# Autodesk Inventor assembly: construction
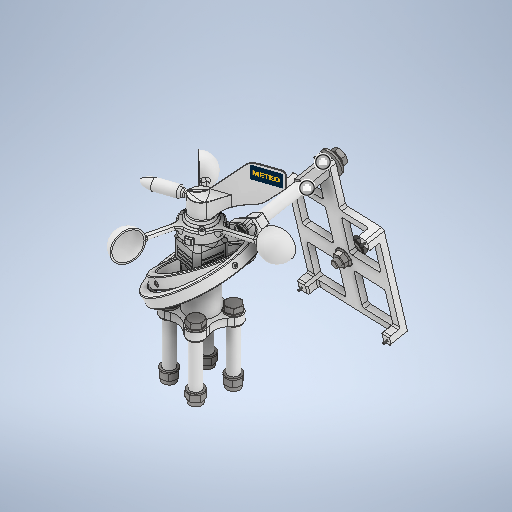
[picture p0: Inventor's stored thumbnail of the model, 512x512]
Saved by Autodesk Inventor 2025.2 (Build 292293000, 293)
## iProperties
Created: 2025-02-10
Part Number: construction
Document SubType Name: Assembly
Designer: yehorderehus
Mass: 762.848 g
Surface Area: 1512.83 cm^2
Volume: 321.338 cm^3
Density: 2.37397 g/cm^3
Author: yehorderehus
## Documents named in this file (32)
- G:\.shortcut-targets-by-id\1Afqr12NmjXaFk11r_F7oLitoDl4TiMfc\Structures\assembly\assembly.iam
- G:\.shortcut-targets-by-id\1Afqr12NmjXaFk11r_F7oLitoDl4TiMfc\Structures\assembly\base-radiator.ipt
- G:\.shortcut-targets-by-id\1Afqr12NmjXaFk11r_F7oLitoDl4TiMfc\Structures\assembly\connector-main.ipt
- G:\.shortcut-targets-by-id\1Afqr12NmjXaFk11r_F7oLitoDl4TiMfc\Structures\assembly\magnet-holder.ipt
- G:\.shortcut-targets-by-id\1Afqr12NmjXaFk11r_F7oLitoDl4TiMfc\Structures\assembly\assets\skf_bearing_623-2z_2.iam
- G:\.shortcut-targets-by-id\1Afqr12NmjXaFk11r_F7oLitoDl4TiMfc\Structures\assembly\assets\skf_bearing_608-2z_2.iam
- G:\.shortcut-targets-by-id\1Afqr12NmjXaFk11r_F7oLitoDl4TiMfc\Structures\assembly\speed-rotor.ipt
- G:\.shortcut-targets-by-id\1Afqr12NmjXaFk11r_F7oLitoDl4TiMfc\Structures\assembly\distance-ring.ipt
- G:\.shortcut-targets-by-id\1Afqr12NmjXaFk11r_F7oLitoDl4TiMfc\Structures\assembly\bearing-clamp.ipt
- G:\.shortcut-targets-by-id\1Afqr12NmjXaFk11r_F7oLitoDl4TiMfc\Structures\assembly\direction-vane.ipt
- G:\.shortcut-targets-by-id\1Afqr12NmjXaFk11r_F7oLitoDl4TiMfc\Structures\assembly\Ambient_board_Meteostanice.iam
- G:\.shortcut-targets-by-id\1Afqr12NmjXaFk11r_F7oLitoDl4TiMfc\Structures\assembly\o-ring.ipt
- G:\.shortcut-targets-by-id\1Afqr12NmjXaFk11r_F7oLitoDl4TiMfc\Structures\assembly\i-ring.ipt
- D:\Users\yehorderehus\Documents\Inventor\Content Center Files\R2025\en-US\ISO 4014(2)\ISO 4014 - M12 x 90 - ISO.ipt
- D:\Users\yehorderehus\Documents\Inventor\Content Center Files\R2025\en-US\DIN 7985 (H)\DIN 7985 (H) - M3x5-H.ipt
- D:\Users\yehorderehus\Documents\Inventor\Content Center Files\R2025\en-US\DIN 7985 (H)\DIN 7985 (H) - M3x16-H.ipt
- D:\Users\yehorderehus\Documents\Inventor\Content Center Files\R2025\en-US\SFS 2976\SFS 2976 - M3 x 40.ipt
- G:\.shortcut-targets-by-id\1Afqr12NmjXaFk11r_F7oLitoDl4TiMfc\Structures\assembly\assets\magnet5_2.ipt
- G:\.shortcut-targets-by-id\1Afqr12NmjXaFk11r_F7oLitoDl4TiMfc\Structures\assembly\assets\magnet10_5.ipt
- G:\.shortcut-targets-by-id\1Afqr12NmjXaFk11r_F7oLitoDl4TiMfc\Structures\assembly\m12-60-ring.ipt
- G:\.shortcut-targets-by-id\1Afqr12NmjXaFk11r_F7oLitoDl4TiMfc\Structures\assembly\assets\Hexagon nut DIN 6334 M10 51103_100_040(High).ipt
- G:\.shortcut-targets-by-id\1Afqr12NmjXaFk11r_F7oLitoDl4TiMfc\Structures\assembly\box-mount.ipt
- D:\Users\yehorderehus\Documents\Inventor\Content Center Files\R2025\en-US\DIN 9021\DIN 9021 - 10,5.ipt
- D:\Users\yehorderehus\Documents\Inventor\Content Center Files\R2025\en-US\DIN 128\DIN 128 - A10.ipt
- D:\Users\yehorderehus\Documents\Inventor\Content Center Files\R2025\en-US\DIN 933\DIN 933 - M10  x 30.ipt
- D:\Users\yehorderehus\Documents\Inventor\Content Center Files\R2025\en-US\ISO 7380-1\ISO 7380-1 - M10 x 90.ipt
- D:\Users\yehorderehus\Documents\Inventor\Content Center Files\R2025\en-US\DIN 6923\DIN 6923 - M10 x 1,5.ipt
- D:\Users\yehorderehus\Documents\Inventor\Content Center Files\R2025\en-US\ISO 7045  H\ISO 7045 - M3 x 25_ - 4.8 - H - ISO.ipt
- G:\.shortcut-targets-by-id\1Afqr12NmjXaFk11r_F7oLitoDl4TiMfc\Structures\assembly\m10-52-ring.ipt
- D:\Users\yehorderehus\Documents\Inventor\Content Center Files\R2025\en-US\ISO 7092\ISO 7092 - ST 12 - 140 HV.ipt
- G:\.shortcut-targets-by-id\1Afqr12NmjXaFk11r_F7oLitoDl4TiMfc\Structures\assembly\assets\insert_m3_5-7.ipt
- D:\Users\yehorderehus\Documents\Inventor\Content Center Files\R2025\en-US\ISO 10512\ISO 10512 - M12 x 1,5.ipt
## Components (81 placed, 31 different names)
1. connector-main:1 — Mate:1, Rotational:1, Flush:1, Flush:2, Rotational:10, Flush:3, Rigid:25, Rigid:4, Rotational:50, Rotational:51, Rigid:55, Rigid:56, Rigid:57, Rigid:58, Rigid:59, Rigid:60, Rigid:61, Rigid:64
2. base-radiator:1 — Rotational:1, Flush:1, Rotational:2, Rotational:4, Rotational:8, Rigid:33, Rigid:32, Rigid:31
3. magnet-holder:1 — Rotational:3, Rotational:12, Rigid:30
4. distance-ring:1 — Rotational:6, Rotational:7
5. bearing-clamp:1 — Rotational:8
6. direction-vane:1 — Rotational:9, Rigid:37
7. speed-rotor:1 — Rigid:35, Rigid:34, Rigid:36, Rigid:29, Rotational:5
8. o-ring:1 — Rigid:26, Rigid:27, Rotational:24, Rigid:62, Rigid:63
9. i-ring:1 — Rotational:25, Rigid:50, Rigid:54
10. Ambient_board_Meteostanice:1 [sub-assembly] — Rotational:10, Flush:3, Rigid:1, Rigid:2, Rigid:3
11. skf_bearing_623-2z_2:1 [sub-assembly] — Rotational:2, Rotational:3
12. skf_bearing_608-2z_2:1 [sub-assembly] — Rotational:4, Rotational:5, Rotational:6
13. skf_bearing_608-2z_2:2 [sub-assembly] — Rotational:7, Rotational:9
14. magnet10_5:1 — Rigid:30
15. SFS 2976 M3 x 40:1 — Rotational:12
16. DIN 7985 (H) M3x16-H:1 — Rigid:27
17. DIN 7985 (H) M3x16-H:2 — Rigid:26, Rotational:25
18. SFS 2976 M3 x 40:2 — Rigid:25, Rotational:24
19. SFS 2976 M3 x 40:3 — Rigid:4
20. DIN 7985 (H) M3x5-H:1 — Rigid:33
21. DIN 7985 (H) M3x5-H:2 — Rigid:32
22. DIN 7985 (H) M3x5-H:3 — Rigid:31
23. DIN 7985 (H) M3x5-H:4 — Rigid:35
24. DIN 7985 (H) M3x5-H:5 — Rigid:34
25. DIN 7985 (H) M3x5-H:6 — Rigid:36
26. DIN 7985 (H) M3x5-H:7 — Rigid:37
27. DIN 7985 (H) M3x5-H:8 — Rigid:3
28. DIN 7985 (H) M3x5-H:9 — Rigid:1
29. DIN 7985 (H) M3x5-H:10 — Rigid:2
30. ISO 7380-1 M10 x 90:1 — Rigid:50, Rigid:52
31. m10-52-ring:1 — Rigid:54
32. Hexagon nut DIN 6334 M10 51103_100_040(High):1 — Rigid:49
33. box-mount:1 — Rigid:46, Rotational:48, Rigid:49, Mate:15, Rigid:53, Angle:1
34. DIN 933 - replaced by DIN EN 24017 M10  x 30:1 — Mate:4, Mate:5, Mate:8, Rigid:52
35. DIN 9021 10,5:1 — Mate:4, Mate:5, Mate:9
36. DIN 128 A10:1 — Mate:8, Mate:9, Rotational:48
37. DIN 933 - replaced by DIN EN 24017 M10  x 30:2 — Mate:6, Mate:7, Mate:12, Mate:14
38. DIN 9021 10,5:2 — Mate:6, Mate:7, Mate:13
39. DIN 128 A10:2 — Mate:12, Mate:13, Rigid:46
40. DIN 6923 M10:1 — Mate:14, Mate:15
41. insert_m3_5-7:1 — Rigid:55
42. insert_m3_5-7:2 — Rigid:56
43. insert_m3_5-7:3 — Rigid:57
44. insert_m3_5-7:4 — Rigid:61
45. insert_m3_5-7:5 — Rigid:58
46. insert_m3_5-7:6 — Rigid:59
47. insert_m3_5-7:7 — Rigid:60
48. insert_m3_5-7:8 — Rigid:64
49. insert_m3_5-7:9 — Rigid:62
50. insert_m3_5-7:10 — Rigid:63
51. magnet5_2:1 — Rigid:29
52. magnet5_2:2
53. magnet5_2:3
54. ISO 4014 M12 x 90:5 — Rotational:49, Rotational:54
55. ISO 7092 ST 12 - 140 HV:1 — Rotational:49, Rotational:50
56. ISO 7092 ST 12 - 140 HV:2 — Rotational:51, Rotational:52
57. m12-60-ring:1 — Rotational:52, Rotational:53
58. ISO 7092 ST 12 - 140 HV:3 — Rotational:53
59. DIN EN ISO 10512 M12 x 1,5:1 — Rotational:54
60. ISO 4014 M12 x 90:6
61. ISO 7092 ST 12 - 140 HV:4
62. ISO 7092 ST 12 - 140 HV:5
63. m12-60-ring:2
64. ISO 7092 ST 12 - 140 HV:6
65. DIN EN ISO 10512 M12 x 1,5:2
66. ISO 4014 M12 x 90:7
67. ISO 7092 ST 12 - 140 HV:7
68. ISO 7092 ST 12 - 140 HV:8
69. m12-60-ring:3
70. ISO 7092 ST 12 - 140 HV:9
71. DIN EN ISO 10512 M12 x 1,5:3
72. ISO 4014 M12 x 90:8
73. ISO 7092 ST 12 - 140 HV:10
74. ISO 7092 ST 12 - 140 HV:11
75. m12-60-ring:4
76. ISO 7092 ST 12 - 140 HV:12
77. DIN EN ISO 10512 M12 x 1,5:4
78. ISO 7045 H M3 x 25 - 4.8 - H:1 — Rigid:53
79. ISO 7045 H M3 x 25 - 4.8 - H:2
80. ISO 7045 H M3 x 25 - 4.8 - H:3
81. ISO 7045 H M3 x 25 - 4.8 - H:4
## Component patterns: (3 elements, first: magnet5_2:1), (4 elements, first: ISO 4014 M12 x 90:5 + ISO 7092 ST 12 - 140 HV:1 + ISO 7092 ST 12 - 140 HV:2 + m12-60-ring:1 + ISO 7092 ST 12 - 140 HV:3 + DIN EN ISO 10512 M12 x 1,5:1), (4 elements, first: ISO 7045 H M3 x 25 - 4.8 - H:1)
## Relationships (67: WeldJoint 32, RevoluteJoint 20, Mate 11, Flush 3, Angle 1)
- Mate:1: connector-main:1
- Rotational:1 [RevoluteJoint]: connector-main:1 ↔ base-radiator:1
- Flush:1: connector-main:1 ↔ base-radiator:1
- Rotational:2 [RevoluteJoint]: base-radiator:1 ↔ skf_bearing_623-2z_2:1
- Rotational:3 [RevoluteJoint]: magnet-holder:1 ↔ skf_bearing_623-2z_2:1
- Rotational:4 [RevoluteJoint]: base-radiator:1 ↔ skf_bearing_608-2z_2:1
- Rotational:6 [RevoluteJoint]: distance-ring:1 ↔ skf_bearing_608-2z_2:1
- Rotational:7 [RevoluteJoint]: distance-ring:1 ↔ skf_bearing_608-2z_2:2
- Flush:2 (61.038 mm): connector-main:1
- Rotational:8 [RevoluteJoint]: base-radiator:1 ↔ bearing-clamp:1
- Rotational:9 [RevoluteJoint]: direction-vane:1 ↔ skf_bearing_608-2z_2:2
- Rotational:10 [RevoluteJoint]: connector-main:1 ↔ Ambient_board_Meteostanice:1
- Flush:3 (1.8 mm): connector-main:1 ↔ Ambient_board_Meteostanice:1
- Rotational:12 [RevoluteJoint]: magnet-holder:1 ↔ SFS 2976 M3 x 40:1
- Rigid:33 [WeldJoint]: base-radiator:1 ↔ DIN 7985 (H) M3x5-H:1
- Rigid:32 [WeldJoint]: base-radiator:1 ↔ DIN 7985 (H) M3x5-H:2
- Rigid:31 [WeldJoint]: base-radiator:1 ↔ DIN 7985 (H) M3x5-H:3
- Rigid:35 [WeldJoint] (0.2 mm): speed-rotor:1 ↔ DIN 7985 (H) M3x5-H:4
- Rigid:34 [WeldJoint] (0.2 mm): speed-rotor:1 ↔ DIN 7985 (H) M3x5-H:5
- Rigid:36 [WeldJoint] (0.2 mm): speed-rotor:1 ↔ DIN 7985 (H) M3x5-H:6
- Rigid:37 [WeldJoint] (0.4 mm): direction-vane:1 ↔ DIN 7985 (H) M3x5-H:7
- Rigid:1 [WeldJoint]: Ambient_board_Meteostanice:1 ↔ DIN 7985 (H) M3x5-H:9
- Rigid:2 [WeldJoint]: Ambient_board_Meteostanice:1 ↔ DIN 7985 (H) M3x5-H:10
- Rigid:3 [WeldJoint]: Ambient_board_Meteostanice:1 ↔ DIN 7985 (H) M3x5-H:8
- Rigid:25 [WeldJoint]: connector-main:1 ↔ SFS 2976 M3 x 40:2
- Rigid:4 [WeldJoint]: connector-main:1 ↔ SFS 2976 M3 x 40:3
- Rigid:26 [WeldJoint]: o-ring:1 ↔ DIN 7985 (H) M3x16-H:2
- Rigid:27 [WeldJoint]: o-ring:1 ↔ DIN 7985 (H) M3x16-H:1
- Rotational:24 [RevoluteJoint] (-0.4 mm): o-ring:1 ↔ SFS 2976 M3 x 40:2
- Rotational:25 [RevoluteJoint] (0.4 mm): i-ring:1 ↔ DIN 7985 (H) M3x16-H:2
- Rigid:29 [WeldJoint]: speed-rotor:1 ↔ magnet5_2:1
- Rotational:5 [RevoluteJoint]: speed-rotor:1 ↔ skf_bearing_608-2z_2:1
- Rigid:30 [WeldJoint]: magnet-holder:1 ↔ magnet10_5:1
- Mate:4: DIN 933 - replaced by DIN EN 24017 M10  x 30:1 ↔ DIN 9021 10,5:1
- Mate:5 (4.2 mm): DIN 933 - replaced by DIN EN 24017 M10  x 30:1 ↔ DIN 9021 10,5:1
- Mate:6: DIN 933 - replaced by DIN EN 24017 M10  x 30:2 ↔ DIN 9021 10,5:2
- Mate:7 (4.2 mm): DIN 933 - replaced by DIN EN 24017 M10  x 30:2 ↔ DIN 9021 10,5:2
- Mate:8: DIN 933 - replaced by DIN EN 24017 M10  x 30:1 ↔ DIN 128 A10:1
- Mate:9 (0.2 mm): DIN 9021 10,5:1 ↔ DIN 128 A10:1
- Mate:12: DIN 933 - replaced by DIN EN 24017 M10  x 30:2 ↔ DIN 128 A10:2
- Mate:13 (0.2 mm): DIN 9021 10,5:2 ↔ DIN 128 A10:2
- Rigid:46 [WeldJoint] (0.2 mm): box-mount:1 ↔ DIN 128 A10:2
- Rotational:48 [RevoluteJoint] (0.2 mm): box-mount:1 ↔ DIN 128 A10:1
- Rigid:49 [WeldJoint]: Hexagon nut DIN 6334 M10 51103_100_040(High):1 ↔ box-mount:1
- Rigid:50 [WeldJoint]: i-ring:1 ↔ ISO 7380-1 M10 x 90:1
- Rigid:52 [WeldJoint]: ISO 7380-1 M10 x 90:1 ↔ DIN 933 - replaced by DIN EN 24017 M10  x 30:1
- Mate:14: DIN 933 - replaced by DIN EN 24017 M10  x 30:2 ↔ DIN 6923 M10:1
- Mate:15: box-mount:1 ↔ DIN 6923 M10:1
- Rigid:53 [WeldJoint]: box-mount:1 ↔ ISO 7045 H M3 x 25 - 4.8 - H:1
- Angle:1 (-90 deg): box-mount:1
- Rigid:54 [WeldJoint]: i-ring:1 ↔ m10-52-ring:1
- Rotational:49 [RevoluteJoint]: ISO 4014 M12 x 90:5 ↔ ISO 7092 ST 12 - 140 HV:1
- Rotational:50 [RevoluteJoint]: connector-main:1 ↔ ISO 7092 ST 12 - 140 HV:1
- Rotational:51 [RevoluteJoint]: connector-main:1 ↔ ISO 7092 ST 12 - 140 HV:2
- Rotational:52 [RevoluteJoint]: ISO 7092 ST 12 - 140 HV:2 ↔ m12-60-ring:1
- Rotational:53 [RevoluteJoint]: m12-60-ring:1 ↔ ISO 7092 ST 12 - 140 HV:3
- Rotational:54 [RevoluteJoint]: ISO 4014 M12 x 90:5 ↔ DIN EN ISO 10512 M12 x 1,5:1
- Rigid:55 [WeldJoint]: connector-main:1 ↔ insert_m3_5-7:1
- Rigid:56 [WeldJoint]: connector-main:1 ↔ insert_m3_5-7:2
- Rigid:57 [WeldJoint]: connector-main:1 ↔ insert_m3_5-7:3
- Rigid:58 [WeldJoint]: connector-main:1 ↔ insert_m3_5-7:5
- Rigid:59 [WeldJoint]: connector-main:1 ↔ insert_m3_5-7:6
- Rigid:60 [WeldJoint]: connector-main:1 ↔ insert_m3_5-7:7
- Rigid:61 [WeldJoint]: connector-main:1 ↔ insert_m3_5-7:4
- Rigid:62 [WeldJoint]: o-ring:1 ↔ insert_m3_5-7:9
- Rigid:63 [WeldJoint]: o-ring:1 ↔ insert_m3_5-7:10
- Rigid:64 [WeldJoint]: connector-main:1 ↔ insert_m3_5-7:8
